# Autodesk Inventor assembly: Моторный блок
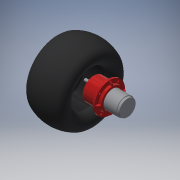
[picture p0: Inventor's stored thumbnail of the model, 180x180]
Saved by Autodesk Inventor 2019 (Build 230136000, 136)
## iProperties
Created: 2022-02-24
Part Number: Моторный блок
Material: Типовые
Document SubType Name: Assembly
Designer: korsh
Author: korsh
## Documents named in this file (5)
- C:\Users\korsh\Desktop\Новая папка (7)\Моторный блок.iam
- C:\Users\korsh\Desktop\Новая папка (7)\mot37.ipt
- C:\Users\korsh\Desktop\Новая папка (7)\Шина.0002.ipt
- C:\Users\korsh\Desktop\Новая папка (7)\Диск.0001.ipt
- C:\Users\korsh\Desktop\Новая папка (7)\Двигатель.ipt
## Components (4 placed, 4 different names)
1. mot37:1 — Совмещение:2, Совмещение:3, Совмещение:4
2. Шина.0002:1 — Совмещение:1
3. Диск.0001:1 — Совмещение:1, Совмещение:2, Совмещение:3
4. Двигатель:1 — Совмещение:4
## Relationships (4: Mate 4)
- Совмещение:1 [Mate]: Шина.0002:1 ↔ Диск.0001:1
- Совмещение:2 [Mate]: mot37:1 ↔ Диск.0001:1
- Совмещение:3 [Mate] (50 mm): mot37:1 ↔ Диск.0001:1
- Совмещение:4 [Mate]: mot37:1 ↔ Двигатель:1
